# Autodesk Inventor assembly: Prototype-PALP-34pipe-with-flange
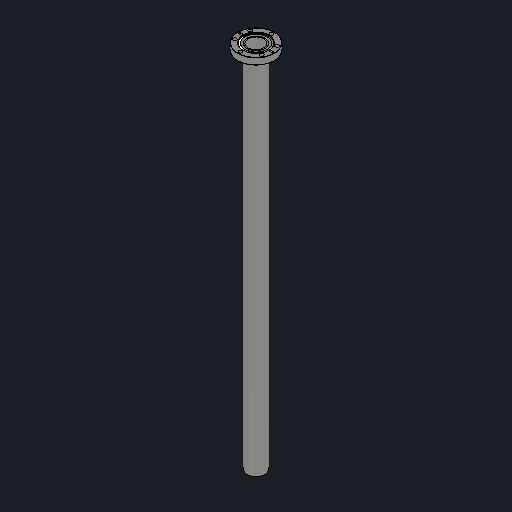
[picture p0: Inventor's stored thumbnail of the model, 512x512]
Saved by Autodesk Inventor 2026 (Build 300175050, 175E)
## iProperties
Created: 2024-05-30
Part Number: Prototype-PALP-34pipe-with-flange
Document SubType Name: Assembly
Designer: kuzmin
Author: kuzmin
## Documents named in this file (3)
- C:\Users\queez\Dropbox\Drawings\PIHTI\PALP\Prototype-PALP-34pipe-with-flange.iam
- C:\Users\queez\Dropbox\Drawings\PIHTI\PALP\Prototype-PALP-34mm-main-pipe.ipt
- C:\Users\queez\Dropbox\Drawings\PIHTI\PALP\Prototype-PALP-CF70-34-hole-flange.ipt
## Components (2 placed, 2 different names)
1. Prototype-PALP-34mm-main-pipe:1
2. Prototype-PALP-CF70-34-hole-flange:1
## Relationships (1: WeldJoint 1)
- [WeldJoint]: Prototype-PALP-34mm-main-pipe:1 ↔ Prototype-PALP-CF70-34-hole-flange:1
